# Autodesk Inventor assembly: 05-22-2023 assieme flangia-verga-curva
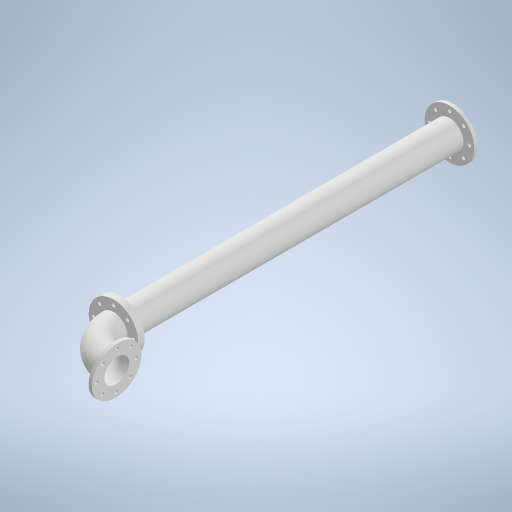
[picture p0: Inventor's stored thumbnail of the model, 512x512]
Saved by Autodesk Inventor 2023 (Build 270158000, 158)
## iProperties
Created: 2023-05-22
Part Number: 05-22-2023 assieme flangia-verga-curva
Document SubType Name: Assembly
Designer: Admin
Author: Admin
## Documents named in this file (4)
- C:\Users\Admin\Desktop\3DDDD\05-22-2023 assieme flangia-verga-curva.iam
- C:\Users\Admin\Desktop\3DDDD\05-22-2023 flangia.ipt
- C:\Users\Admin\Desktop\3DDDD\05-22-2023 verga.ipt
- C:\Users\Admin\Desktop\3DDDD\05-22-2023 curva Sweep.ipt
## Components (6 placed, 3 different names)
1. 05-22-2023 flangia:1 — Coincidente:1, Coincidente:2, Coincidente:3, Coincidente:6
2. 05-22-2023 verga:1 — Coincidente:1, Coincidente:2, Coincidente:3, Coincidente:4, Coincidente:5
3. 05-22-2023 flangia:2 — Coincidente:4, Coincidente:5, Coincidente:6, Coincidente:11, Coincidente:12, Coincidente:13
4. 05-22-2023 curva Sweep:1 — Coincidente:7, Coincidente:8, Coincidente:9, Coincidente:10
5. 05-22-2023 flangia:3 — Coincidente:7, Coincidente:8, Coincidente:11, Coincidente:12, Coincidente:13
6. 05-22-2023 flangia:4 — Coincidente:9, Coincidente:10
## Relationships (13: Mate 13)
- Coincidente:1 [Mate]: 05-22-2023 flangia:1 ↔ 05-22-2023 verga:1
- Coincidente:2 [Mate]: 05-22-2023 flangia:1 ↔ 05-22-2023 verga:1
- Coincidente:3 [Mate]: 05-22-2023 flangia:1 ↔ 05-22-2023 verga:1
- Coincidente:4 [Mate]: 05-22-2023 verga:1 ↔ 05-22-2023 flangia:2
- Coincidente:5 [Mate]: 05-22-2023 verga:1 ↔ 05-22-2023 flangia:2
- Coincidente:6 [Mate]: 05-22-2023 flangia:1 ↔ 05-22-2023 flangia:2
- Coincidente:7 [Mate]: 05-22-2023 curva Sweep:1 ↔ 05-22-2023 flangia:3
- Coincidente:8 [Mate]: 05-22-2023 curva Sweep:1 ↔ 05-22-2023 flangia:3
- Coincidente:9 [Mate]: 05-22-2023 curva Sweep:1 ↔ 05-22-2023 flangia:4
- Coincidente:10 [Mate]: 05-22-2023 curva Sweep:1 ↔ 05-22-2023 flangia:4
- Coincidente:11 [Mate]: 05-22-2023 flangia:2 ↔ 05-22-2023 flangia:3
- Coincidente:12 [Mate]: 05-22-2023 flangia:2 ↔ 05-22-2023 flangia:3
- Coincidente:13 [Mate]: 05-22-2023 flangia:2 ↔ 05-22-2023 flangia:3
